# Autodesk Inventor assembly: 200-40-BOGIE-CONNECTOR-ASM-01
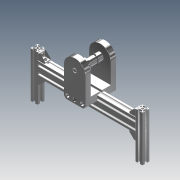
[picture p0: Inventor's stored thumbnail of the model, 180x180]
Saved by Autodesk Inventor 2018.2 (Build 222227000, 227)
## iProperties
Manager: feesmrt
Company: FRANC0R
Created: 2017-12-10
Part Number: 200-40-BOGIE-CONNECTOR-ASM-01
Material: Generisch
Document SubType Name: Assembly
Designer: feesmrt
Project: Rescue Robot
Cost Center: -
Description: Bogie Connector Assembly
Engineer: feesmrt
Authority: feesmrt
Stock Number: 200-40-BOGIE-CONNECTOR-ASM-01
Mass: 975.454 g
Surface Area: 1626.6 cm^2
Volume: 351.256 cm^3
Density: 2.77705 g/cm^3
Author: feesmrt
Title: Bogie Connector Assembly
Subject: Rescue Robot
Revision Number: 1
## Documents named in this file (11)
- D:\Programmierung\FRANC0R\CAD\02-Rocker-Bogie-Robot\200-ROCKER-BOGIE\200-40-BOGIE-CONNECTOR\200-40-BOGIE-CONNECTOR-ASM-01.iam
- D:\Programmierung\FRANC0R\CAD\02-Rocker-Bogie-Robot\200-ROCKER-BOGIE\200-40-BOGIE-CONNECTOR\200-40-BOGIE-CONNECTOR-05.ipt
- D:\Programmierung\FRANC0R\CAD\02-Rocker-Bogie-Robot\200-ROCKER-BOGIE\200-40-BOGIE-CONNECTOR\200-40-BOGIE-CONNECTOR-03.ipt
- D:\Programmierung\FRANC0R\CAD\02-Rocker-Bogie-Robot\200-ROCKER-BOGIE\200-40-BOGIE-CONNECTOR\200-40-BOGIE-CONNECTOR-04.ipt
- D:\Programmierung\FRANC0R\CAD\02-Rocker-Bogie-Robot\900-COMPONENTS\900-40-SCREWS\900-40-SCREWS-DIN7984_M5x25.ipt
- D:\Programmierung\FRANC0R\CAD\02-Rocker-Bogie-Robot\900-COMPONENTS\900-40-SCREWS\900-40-SCREWS-DIN7984_M5x12.ipt
- D:\Programmierung\FRANC0R\CAD\02-Rocker-Bogie-Robot\900-COMPONENTS\900-50-PROFILES\900-50-PROFILES-CONN-N6xM5.ipt
- D:\Programmierung\FRANC0R\CAD\02-Rocker-Bogie-Robot\900-COMPONENTS\900-60-CIRCLIPS\900-60-CIRCLIPS-DIN471-20x1,2.ipt
- D:\Programmierung\FRANC0R\CAD\02-Rocker-Bogie-Robot\200-ROCKER-BOGIE\200-40-BOGIE-CONNECTOR\200-40-BOGIE-CONNECTOR-P-01.ipt
- D:\Programmierung\FRANC0R\CAD\02-Rocker-Bogie-Robot\200-ROCKER-BOGIE\200-40-BOGIE-CONNECTOR\200-40-BOGIE-CONNECTOR-P-02.ipt
- D:\Programmierung\FRANC0R\CAD\02-Rocker-Bogie-Robot\900-COMPONENTS\900-50-PROFILES\900-50-PROFILES-ANGLE-CONN-20x20-01.iam
## Components (23 placed, 10 different names)
1. 200-40-BOGIE-CONNECTOR-05:1 — Passend:6, Passend:7, Fluchtend:7, Passend:8, Passend:9, Passend:10, Passend:45, Passend:46
2. 200-40-BOGIE-CONNECTOR-03:2 — Passend:8, Passend:9, Passend:10, Passend:16, Fluchtend:10, Passend:23, Passend:25, Passend:34, Passend:35
3. 200-40-BOGIE-CONNECTOR-03:1 — Passend:6, Passend:7, Fluchtend:7, Passend:17, Passend:24, Fluchtend:11, Passend:33, Passend:36
4. 200-40-BOGIE-CONNECTOR-04:1 — Passend:17, Passend:24, Fluchtend:11, Passend:29, Passend:30, Passend:31, Passend:32, Passend:39, Passend:40, Winkel:1, Winkel:2, Passend:49
5. 200-40-BOGIE-CONNECTOR-04:2 — Passend:16, Fluchtend:10, Passend:23, Passend:26, Passend:27, Passend:28, Passend:37, Passend:38, Winkel:3, Winkel:4
6. 900-40-SCREWS-DIN7984_M5x25:1 — Passend:25, Passend:26, Passend:41
7. 900-40-SCREWS-DIN7984_M5x25:2 — Passend:27, Passend:28, Passend:42
8. 900-40-SCREWS-DIN7984_M5x25:3 — Passend:30, Passend:32, Passend:44
9. 900-40-SCREWS-DIN7984_M5x25:4 — Passend:29, Passend:31, Passend:43
10. 900-40-SCREWS-DIN7984_M5x12:1 — Passend:33, Passend:36
11. 900-40-SCREWS-DIN7984_M5x12:2 — Passend:34, Passend:35
12. 900-50-PROFILES-CONN-N6xM5:1 — Passend:37, Passend:42, Winkel:4
13. 900-50-PROFILES-CONN-N6xM5:2 — Passend:38, Passend:41, Winkel:3
14. 900-50-PROFILES-CONN-N6xM5:3 — Passend:40, Passend:44, Winkel:2
15. 900-50-PROFILES-CONN-N6xM5:4 — Passend:39, Passend:43, Winkel:1
16. 900-60-CIRCLIPS-DIN471-20x1,2:1 — Passend:45, Passend:46, Fluchtend:12
17. 200-40-BOGIE-CONNECTOR-P-01:1 — Passend:47, Passend:48, Passend:49, Fluchtend:13, Fluchtend:14, Fluchtend:15, Fluchtend:16, Passend:50, Passend:51, Passend:52, Passend:54, Passend:57, Passend:60, Passend:61
18. 200-40-BOGIE-CONNECTOR-P-02:1 — Fluchtend:13, Fluchtend:15, Passend:50, Passend:53, Passend:59, Passend:63
19. 200-40-BOGIE-CONNECTOR-P-02:2 — Fluchtend:14, Fluchtend:16, Passend:51, Passend:55, Passend:56, Passend:58, Passend:62
20. 900-50-PROFILES-ANGLE-CONN-20x20-01:1 [sub-assembly] — Passend:52, Passend:53, Passend:57
21. 900-50-PROFILES-ANGLE-CONN-20x20-01:2 [sub-assembly] — Passend:54, Passend:55, Passend:56
22. 900-50-PROFILES-ANGLE-CONN-20x20-01:3 [sub-assembly] — Passend:58, Passend:61, Passend:62
23. 900-50-PROFILES-ANGLE-CONN-20x20-01:4 [sub-assembly] — Passend:59, Passend:60, Passend:63
## Relationships (60: Mate 48, Flush 8, Angle 4)
- Passend:6 [Mate]: 200-40-BOGIE-CONNECTOR-05:1 ↔ 200-40-BOGIE-CONNECTOR-03:1
- Passend:7 [Mate]: 200-40-BOGIE-CONNECTOR-05:1 ↔ 200-40-BOGIE-CONNECTOR-03:1
- Fluchtend:7 [Flush]: 200-40-BOGIE-CONNECTOR-05:1 ↔ 200-40-BOGIE-CONNECTOR-03:1
- Passend:8 [Mate]: 200-40-BOGIE-CONNECTOR-05:1 ↔ 200-40-BOGIE-CONNECTOR-03:2
- Passend:9 [Mate]: 200-40-BOGIE-CONNECTOR-05:1 ↔ 200-40-BOGIE-CONNECTOR-03:2
- Passend:10 [Mate]: 200-40-BOGIE-CONNECTOR-05:1 ↔ 200-40-BOGIE-CONNECTOR-03:2
- Passend:16 [Mate]: 200-40-BOGIE-CONNECTOR-03:2 ↔ 200-40-BOGIE-CONNECTOR-04:2
- Passend:17 [Mate]: 200-40-BOGIE-CONNECTOR-03:1 ↔ 200-40-BOGIE-CONNECTOR-04:1
- Fluchtend:10 [Flush]: 200-40-BOGIE-CONNECTOR-03:2 ↔ 200-40-BOGIE-CONNECTOR-04:2
- Passend:23 [Mate]: 200-40-BOGIE-CONNECTOR-03:2 ↔ 200-40-BOGIE-CONNECTOR-04:2
- Passend:24 [Mate]: 200-40-BOGIE-CONNECTOR-03:1 ↔ 200-40-BOGIE-CONNECTOR-04:1
- Fluchtend:11 [Flush]: 200-40-BOGIE-CONNECTOR-03:1 ↔ 200-40-BOGIE-CONNECTOR-04:1
- Passend:25 [Mate]: 200-40-BOGIE-CONNECTOR-03:2 ↔ 900-40-SCREWS-DIN7984_M5x25:1
- Passend:26 [Mate]: 200-40-BOGIE-CONNECTOR-04:2 ↔ 900-40-SCREWS-DIN7984_M5x25:1
- Passend:27 [Mate]: 200-40-BOGIE-CONNECTOR-04:2 ↔ 900-40-SCREWS-DIN7984_M5x25:2
- Passend:28 [Mate]: 200-40-BOGIE-CONNECTOR-04:2 ↔ 900-40-SCREWS-DIN7984_M5x25:2
- Passend:29 [Mate]: 200-40-BOGIE-CONNECTOR-04:1 ↔ 900-40-SCREWS-DIN7984_M5x25:4
- Passend:30 [Mate]: 200-40-BOGIE-CONNECTOR-04:1 ↔ 900-40-SCREWS-DIN7984_M5x25:3
- Passend:31 [Mate]: 200-40-BOGIE-CONNECTOR-04:1 ↔ 900-40-SCREWS-DIN7984_M5x25:4
- Passend:32 [Mate]: 200-40-BOGIE-CONNECTOR-04:1 ↔ 900-40-SCREWS-DIN7984_M5x25:3
- Passend:33 [Mate]: 200-40-BOGIE-CONNECTOR-03:1 ↔ 900-40-SCREWS-DIN7984_M5x12:1
- Passend:34 [Mate]: 200-40-BOGIE-CONNECTOR-03:2 ↔ 900-40-SCREWS-DIN7984_M5x12:2
- Passend:35 [Mate]: 200-40-BOGIE-CONNECTOR-03:2 ↔ 900-40-SCREWS-DIN7984_M5x12:2
- Passend:36 [Mate]: 200-40-BOGIE-CONNECTOR-03:1 ↔ 900-40-SCREWS-DIN7984_M5x12:1
- Passend:37 [Mate] (1.5 mm): 200-40-BOGIE-CONNECTOR-04:2 ↔ 900-50-PROFILES-CONN-N6xM5:1
- Passend:38 [Mate] (1.5 mm): 200-40-BOGIE-CONNECTOR-04:2 ↔ 900-50-PROFILES-CONN-N6xM5:2
- Passend:39 [Mate] (1.5 mm): 200-40-BOGIE-CONNECTOR-04:1 ↔ 900-50-PROFILES-CONN-N6xM5:4
- Passend:40 [Mate] (1.5 mm): 200-40-BOGIE-CONNECTOR-04:1 ↔ 900-50-PROFILES-CONN-N6xM5:3
- Passend:41 [Mate]: 900-40-SCREWS-DIN7984_M5x25:1 ↔ 900-50-PROFILES-CONN-N6xM5:2
- Passend:42 [Mate]: 900-40-SCREWS-DIN7984_M5x25:2 ↔ 900-50-PROFILES-CONN-N6xM5:1
- Passend:43 [Mate]: 900-40-SCREWS-DIN7984_M5x25:4 ↔ 900-50-PROFILES-CONN-N6xM5:4
- Passend:44 [Mate]: 900-40-SCREWS-DIN7984_M5x25:3 ↔ 900-50-PROFILES-CONN-N6xM5:3
- Winkel:1 [Angle] (0 deg): 200-40-BOGIE-CONNECTOR-04:1 ↔ 900-50-PROFILES-CONN-N6xM5:4
- Winkel:2 [Angle] (0 deg): 200-40-BOGIE-CONNECTOR-04:1 ↔ 900-50-PROFILES-CONN-N6xM5:3
- Winkel:3 [Angle] (0 deg): 200-40-BOGIE-CONNECTOR-04:2 ↔ 900-50-PROFILES-CONN-N6xM5:2
- Winkel:4 [Angle] (0 deg): 200-40-BOGIE-CONNECTOR-04:2 ↔ 900-50-PROFILES-CONN-N6xM5:1
- Passend:45 [Mate]: 200-40-BOGIE-CONNECTOR-05:1 ↔ 900-60-CIRCLIPS-DIN471-20x1,2:1
- Passend:46 [Mate]: 200-40-BOGIE-CONNECTOR-05:1 ↔ 900-60-CIRCLIPS-DIN471-20x1,2:1
- Fluchtend:12 [Flush]: 900-60-CIRCLIPS-DIN471-20x1,2:1
- Passend:47 [Mate]: 200-40-BOGIE-CONNECTOR-P-01:1
- Passend:48 [Mate]: 200-40-BOGIE-CONNECTOR-P-01:1
- Passend:49 [Mate]: 200-40-BOGIE-CONNECTOR-04:1 ↔ 200-40-BOGIE-CONNECTOR-P-01:1
- Fluchtend:13 [Flush] (-20 mm): 200-40-BOGIE-CONNECTOR-P-01:1 ↔ 200-40-BOGIE-CONNECTOR-P-02:1
- Fluchtend:14 [Flush] (-20 mm): 200-40-BOGIE-CONNECTOR-P-01:1 ↔ 200-40-BOGIE-CONNECTOR-P-02:2
- Fluchtend:15 [Flush]: 200-40-BOGIE-CONNECTOR-P-01:1 ↔ 200-40-BOGIE-CONNECTOR-P-02:1
- Fluchtend:16 [Flush]: 200-40-BOGIE-CONNECTOR-P-01:1 ↔ 200-40-BOGIE-CONNECTOR-P-02:2
- Passend:50 [Mate]: 200-40-BOGIE-CONNECTOR-P-01:1 ↔ 200-40-BOGIE-CONNECTOR-P-02:1
- Passend:51 [Mate]: 200-40-BOGIE-CONNECTOR-P-01:1 ↔ 200-40-BOGIE-CONNECTOR-P-02:2
- Passend:52 [Mate]: 200-40-BOGIE-CONNECTOR-P-01:1 ↔ 900-50-PROFILES-ANGLE-CONN-20x20-01:1
- Passend:53 [Mate]: 200-40-BOGIE-CONNECTOR-P-02:1 ↔ 900-50-PROFILES-ANGLE-CONN-20x20-01:1
- Passend:54 [Mate]: 200-40-BOGIE-CONNECTOR-P-01:1 ↔ 900-50-PROFILES-ANGLE-CONN-20x20-01:2
- Passend:55 [Mate]: 200-40-BOGIE-CONNECTOR-P-02:2 ↔ 900-50-PROFILES-ANGLE-CONN-20x20-01:2
- Passend:56 [Mate]: 200-40-BOGIE-CONNECTOR-P-02:2 ↔ 900-50-PROFILES-ANGLE-CONN-20x20-01:2
- Passend:57 [Mate]: 200-40-BOGIE-CONNECTOR-P-01:1 ↔ 900-50-PROFILES-ANGLE-CONN-20x20-01:1
- Passend:58 [Mate]: 200-40-BOGIE-CONNECTOR-P-02:2 ↔ 900-50-PROFILES-ANGLE-CONN-20x20-01:3
- Passend:59 [Mate]: 200-40-BOGIE-CONNECTOR-P-02:1 ↔ 900-50-PROFILES-ANGLE-CONN-20x20-01:4
- Passend:60 [Mate]: 200-40-BOGIE-CONNECTOR-P-01:1 ↔ 900-50-PROFILES-ANGLE-CONN-20x20-01:4
- Passend:61 [Mate]: 200-40-BOGIE-CONNECTOR-P-01:1 ↔ 900-50-PROFILES-ANGLE-CONN-20x20-01:3
- Passend:62 [Mate]: 200-40-BOGIE-CONNECTOR-P-02:2 ↔ 900-50-PROFILES-ANGLE-CONN-20x20-01:3
- Passend:63 [Mate]: 200-40-BOGIE-CONNECTOR-P-02:1 ↔ 900-50-PROFILES-ANGLE-CONN-20x20-01:4
